# Autodesk Inventor assembly: ArmController
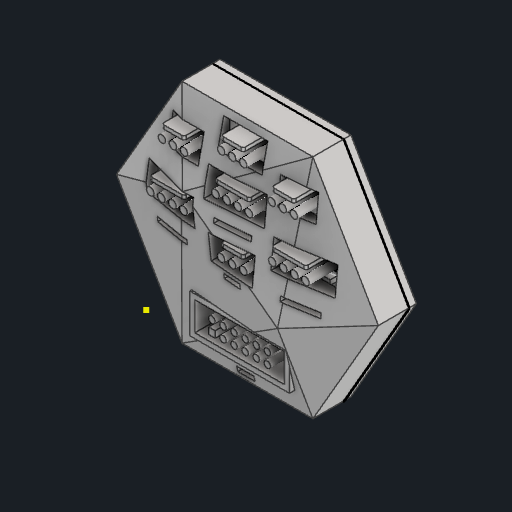
[picture p0: Inventor's stored thumbnail of the model, 512x512]
Saved by Autodesk Inventor 2023 (Build 270158000, 158)
## iProperties
Created: 2023-12-09
Part Number: ArmController
Document SubType Name: Assembly
Designer: valer
Author: valer
## Documents named in this file (3)
- C:\Users\valer\Desktop\str1ker\cad\ArmController.iam
- C:\Users\valer\Desktop\str1ker\cad\external\MotorControl\ArmControlBoardPcb.ipt
- C:\Users\valer\Desktop\str1ker\cad\ArmControlBoardCover.ipt
## Components (2 placed, 2 different names)
1. ArmControlBoardPcb:1 — Mate:1, Mate:2, Angle:1, Flush:1
2. ArmControlBoardCover:1 — Flush:1
## Relationships (4: Mate 2, Angle 1, Flush 1)
- Mate:1: ArmControlBoardPcb:1
- Mate:2: ArmControlBoardPcb:1
- Angle:1 (0 deg): ArmControlBoardPcb:1
- Flush:1: ArmControlBoardPcb:1 ↔ ArmControlBoardCover:1
